# Autodesk Inventor assembly: ROBUSTA
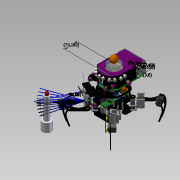
[picture p0: Inventor's stored thumbnail of the model, 180x180]
Saved by Autodesk Inventor 2015 SP1 (Build 190203100, 203)
## iProperties
Created: 2015-02-05
Part Number: ROBUSTA
Document SubType Name: Assembly
Designer: Rafi Kurnia Putra
Author: Rafi Kurnia Putra
## Documents named in this file (11)
- D:\Dropbox\krpai berkaki trui 2015\ROBUSTA\MEKANIK\ROBUSTA\ROBUSTA.iam
- D:\Dropbox\krpai berkaki trui 2015\ROBUSTA\MEKANIK\ROBUSTA\Assembly Base.iam
- D:\Dropbox\krpai berkaki trui 2015\ROBUSTA\MEKANIK\ROBUSTA\Spacer 5cm.ipt
- D:\Dropbox\krpai berkaki trui 2015\ROBUSTA\MEKANIK\ROBUSTA\Box Pengukuran.ipt
- D:\Dropbox\krpai berkaki trui 2015\ROBUSTA\MEKANIK\ROBUSTA\Lapangan.ipt
- D:\Dropbox\krpai berkaki trui 2015\ROBUSTA\MEKANIK\ROBUSTA\Juring Seperempat.ipt
- D:\Dropbox\krpai berkaki trui 2015\ROBUSTA\MEKANIK\ROBUSTA\Lilin.ipt
- D:\Dropbox\krpai berkaki trui 2015\ROBUSTA\MEKANIK\ROBUSTA\Assembly Bumper.iam
- D:\Dropbox\krpai berkaki trui 2015\ROBUSTA\MEKANIK\ROBUSTA\Assembly Kipas.iam
- D:\Dropbox\krpai berkaki trui 2015\ROBUSTA\MEKANIK\ROBUSTA\Assembly Kepala.iam
- D:\Dropbox\krpai berkaki trui 2015\ROBUSTA\MEKANIK\ROBUSTA\Assembly Proximity Servo.iam
## Components (13 placed, 10 different names)
1. Assembly Base:1 [sub-assembly] — Mate:1, Mate:2, Mate:3, Mate:38, Mate:47, Mate:48, Mate:51, Mate:52, Mate:54, Mate:55, Mate:56, Mate:57, Flush:4, Mate:62, Mate:63
2. Box Pengukuran:1 — Flush:4, Mate:62, Mate:63
3. Juring Seperempat:1 — Mate:38, Mate:39, Tangent:1, Tangent:2
4. Lilin:1 — Mate:39, Tangent:1, Tangent:2
5. Assembly Bumper:1 [sub-assembly] — Mate:43, Mate:44, Mate:49, Mate:50, Mate:53, Mate:58, Mate:60, Mate:64, Mate:65, Mate:66, Mate:68
6. Assembly Kipas:1 [sub-assembly] — Mate:43, Mate:44
7. Spacer 5cm:1 — Mate:56, Mate:57
8. Spacer 5cm:2 — Mate:54, Mate:55
9. Spacer 5cm:3 — Mate:51, Mate:52, Mate:53, Mate:59
10. Spacer 5cm:4 — Mate:47, Mate:48, Mate:49, Mate:50
11. Assembly Kepala:1 [sub-assembly] — Mate:58, Mate:59, Mate:60, Flush:2, Flush:3, Angle:1
12. Assembly Proximity Servo:1 [sub-assembly] — Mate:64, Mate:65, Mate:66, Mate:68
13. Lapangan:1 — Mate:67, Angle:1
## Relationships (34: Mate 28, Flush 3, Tangent 2, Angle 1)
- Mate:1: Assembly Base:1
- Mate:2: Assembly Base:1
- Mate:3: Assembly Base:1
- Mate:38 (10 mm): Assembly Base:1 ↔ Juring Seperempat:1
- Mate:39: Juring Seperempat:1 ↔ Lilin:1
- Tangent:1: Juring Seperempat:1 ↔ Lilin:1
- Tangent:2: Juring Seperempat:1 ↔ Lilin:1
- Mate:43: Assembly Bumper:1 ↔ Assembly Kipas:1
- Mate:44: Assembly Bumper:1 ↔ Assembly Kipas:1
- Mate:47: Assembly Base:1 ↔ Spacer 5cm:4
- Mate:48: Assembly Base:1 ↔ Spacer 5cm:4
- Mate:49: Assembly Bumper:1 ↔ Spacer 5cm:4
- Mate:50: Assembly Bumper:1 ↔ Spacer 5cm:4
- Mate:51: Assembly Base:1 ↔ Spacer 5cm:3
- Mate:52: Assembly Base:1 ↔ Spacer 5cm:3
- Mate:53: Assembly Bumper:1 ↔ Spacer 5cm:3
- Mate:54: Assembly Base:1 ↔ Spacer 5cm:2
- Mate:55: Assembly Base:1 ↔ Spacer 5cm:2
- Mate:56: Assembly Base:1 ↔ Spacer 5cm:1
- Mate:57: Assembly Base:1 ↔ Spacer 5cm:1
- Mate:58: Assembly Bumper:1 ↔ Assembly Kepala:1
- Mate:59: Spacer 5cm:3 ↔ Assembly Kepala:1
- Mate:60: Assembly Bumper:1 ↔ Assembly Kepala:1
- Flush:2: Assembly Kepala:1
- Flush:3: Assembly Kepala:1
- Flush:4: Assembly Base:1 ↔ Box Pengukuran:1
- Mate:62: Assembly Base:1 ↔ Box Pengukuran:1
- Mate:63: Assembly Base:1 ↔ Box Pengukuran:1
- Mate:64: Assembly Bumper:1 ↔ Assembly Proximity Servo:1
- Mate:65: Assembly Bumper:1 ↔ Assembly Proximity Servo:1
- Mate:66: Assembly Bumper:1 ↔ Assembly Proximity Servo:1
- Mate:67: Lapangan:1
- Angle:1 (180 deg): Assembly Kepala:1 ↔ Lapangan:1
- Mate:68: Assembly Bumper:1 ↔ Assembly Proximity Servo:1
